# Autodesk Inventor assembly: Right Pulley Stack
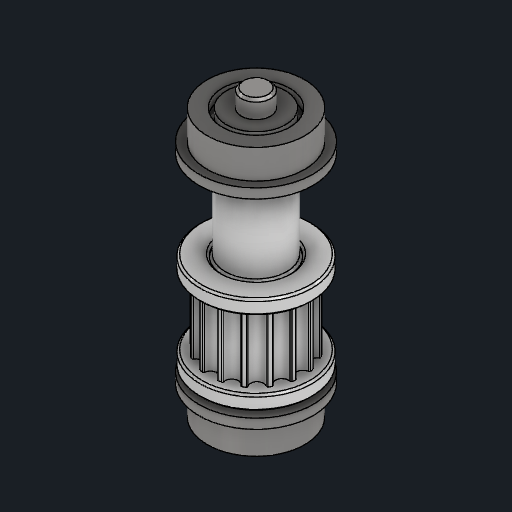
[picture p0: Inventor's stored thumbnail of the model, 512x512]
Saved by Autodesk Inventor 2026.1 (Build 301233020, 233B)
## iProperties
Created: 2025-08-01
Part Number: Right Pulley Stack
Document SubType Name: Assembly
Designer: Joshua Eah
Author: Joshua Eah
## Documents named in this file (6)
- C:\Users\JoshuaEah\Documents\GitHub\Voron-0\CAD\Tulip - Machined Parts\XY Joints\XY Joint Right\Right Pulley Stack.iam
- C:\Users\JoshuaEah\Documents\GitHub\Voron-0\CAD\Master Assembly\Hardware\f623-rs.ipt
- C:\Users\JoshuaEah\Documents\GitHub\Voron-0\CAD\Master Assembly\Hardware\M3_Washer.ipt
- C:\Users\JoshuaEah\Documents\GitHub\Voron-0\CAD\Master Assembly\Hardware\3x30 Pin.ipt
- C:\Users\JoshuaEah\Documents\GitHub\Voron-0\CAD\Machined Parts\Spacers\Spacer.ipt
- C:\Users\JoshuaEah\Documents\GitHub\Voron-0\CAD\Master Assembly\Hardware\GT2 16T 6mm Pulley.ipt
## Components (6 placed, 5 different names)
1. f623-rs:1
2. f623-rs:2
3. M3_Washer:1
4. 3x30 Pin:1
5. Spacer:1
6. 16T_Pulley:1
## Relationships (5: Insert 4, Mate 1)
- [Insert]: f623-rs:1 ↔ M3_Washer:1
- [Insert]: M3_Washer:1 ↔ 16T_Pulley:1
- [Insert]: Spacer:1 ↔ 16T_Pulley:1
- [Insert]: f623-rs:2 ↔ Spacer:1
- [Mate]: 3x30 Pin:1 ↔ 16T_Pulley:1
